# Autodesk Inventor assembly: assembly_v_2_2
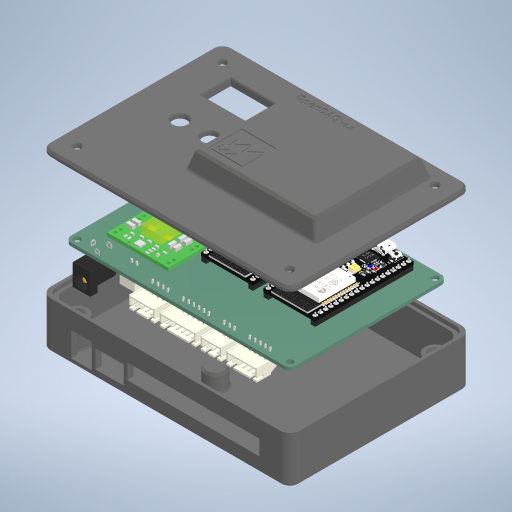
[picture p0: Inventor's stored thumbnail of the model, 512x512]
Saved by Autodesk Inventor 2023 (Build 270158000, 158)
## iProperties
Created: 2023-10-04
Part Number: assembly_v_2_2
Document SubType Name: Assembly
Designer: mark
Author: mark
## Documents named in this file (4)
- D:\Egyetem\BME MSc\Diplomamunka\opendaq\cad\assembly\v_2\assembly_v_2_2.iam
- D:\Egyetem\BME MSc\Diplomamunka\opendaq\cad\housing\v_2\housing_base_v_2.ipt
- D:\Egyetem\BME MSc\Diplomamunka\opendaq\cad\housing\v_2\housing_top_v_2_2.ipt
- D:\Egyetem\BME MSc\Diplomamunka\opendaq\pcb\opendaq_carrier_1.0\opendaq_carrier_1.0.iam
## Components (3 placed, 3 different names)
1. housing_base_v_2:1 — Mate:1, Mate:2, Mate:3, Mate:5, Mate:6
2. housing_top_v_2_2:1 — Mate:4, Mate:5, Mate:6
3. opendaq_carrier_1.0:1 [sub-assembly] — Mate:1, Mate:2, Mate:3, Mate:4
## Relationships (6: Mate 6)
- Mate:1: housing_base_v_2:1 ↔ opendaq_carrier_1.0:1
- Mate:2: housing_base_v_2:1 ↔ opendaq_carrier_1.0:1
- Mate:3 (30 mm): housing_base_v_2:1 ↔ opendaq_carrier_1.0:1
- Mate:4: housing_top_v_2_2:1 ↔ opendaq_carrier_1.0:1
- Mate:5 (60 mm): housing_base_v_2:1 ↔ housing_top_v_2_2:1
- Mate:6: housing_base_v_2:1 ↔ housing_top_v_2_2:1
